# Autodesk Inventor assembly: MG-Chip Kicker
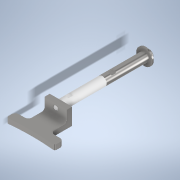
[picture p0: Inventor's stored thumbnail of the model, 180x180]
Saved by Autodesk Inventor 2020 (Build 240168000, 168)
## iProperties
Part Number: MG-Chip Kicker
Material: Generisch
Document SubType Name: Assembly
Designer: rYan
Mass: 43.8833 g
Surface Area: 57.8442 cm^2
Volume: 9.33315 cm^3
Density: 4.70187 g/cm^3
Author: rYan
## Documents named in this file (6)
- D:\github\ssl-mechanics\V2.1(LARC2019)\Inventor\kicker\kicker_assembly_front.iam
- D:\github\ssl-mechanics\V2.1(LARC2019)\Inventor\kicker\kicker_mitte.ipt
- D:\github\ssl-mechanics\V2.1(LARC2019)\Inventor\kicker\kicker_eisen.ipt
- D:\github\ssl-mechanics\V2.1(LARC2019)\Inventor\kicker\compras\DIN 9021 - 6,4.ipt
- D:\github\ssl-mechanics\V2.1(LARC2019)\Inventor\kicker\compras\DIN 7984 - M6 x 10.ipt
- D:\github\ssl-mechanics\V2.1(LARC2019)\Inventor\kicker\kicker_front_head.ipt
## Components (5 placed, 4 different names)
1. Kicker Eisen:1 — Einfügen:1, Rotational:1
2. Kicker Eisen:1 — Einfügen:1, Einfügen:4
3. DIN 9021 6,4:1 — Einfügen:4
4. DIN 7984 M6 x 10:1
5. Kicker Front Head — Rotational:1
## Relationships (4: Insert 3, RevoluteJoint 1)
- Einfügen:1 [Insert]: Kicker Eisen:1
- [Insert]: DIN 9021 6,4:1 ↔ DIN 7984 M6 x 10:1
- Einfügen:4 [Insert]: Kicker Eisen:1 ↔ DIN 9021 6,4:1
- Rotational:1 [RevoluteJoint]: Kicker Eisen:1 ↔ Kicker Front Head
